# Autodesk Inventor assembly: LightRail_assembly
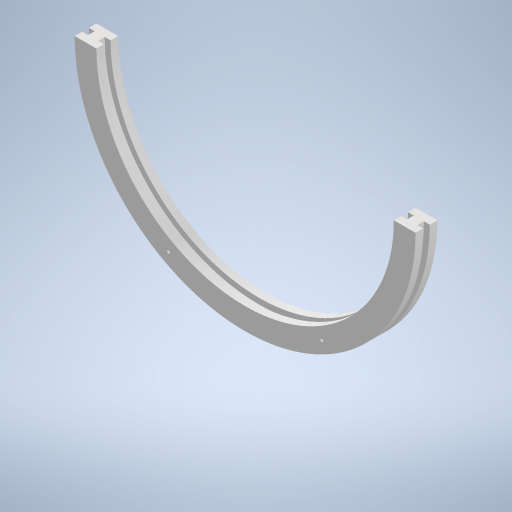
[picture p0: Inventor's stored thumbnail of the model, 512x512]
Saved by Autodesk Inventor 2023 (Build 270158000, 158)
## iProperties
Created: 2023-04-29
Part Number: LightRail_assembly
Document SubType Name: Assembly
Designer: ringl
Author: ringl
## Documents named in this file (3)
- C:\Users\ringl\Documents\Uni Classes\Y3S2\EE318-Project\EE318-Project\CAD\LightRail\LightRail_assembly.iam
- C:\Users\ringl\Documents\Uni Classes\Y3S2\EE318-Project\EE318-Project\CAD\LightRail\LightRail_endSection.ipt
- C:\Users\ringl\Documents\Uni Classes\Y3S2\EE318-Project\EE318-Project\CAD\LightRail\LightRail_middleSection.ipt
## Components (3 placed, 2 different names)
1. LightRail_endSection:1 — Mate:1, Mate:2, Flush:1
2. LightRail_middleSection:1 — Mate:1, Mate:2, Flush:1, Flush:2, Mate:3, Mate:4
3. LightRail_endSection:2 — Flush:2, Mate:3, Mate:4
## Relationships (6: Mate 4, Flush 2)
- Mate:1: LightRail_endSection:1 ↔ LightRail_middleSection:1
- Mate:2: LightRail_endSection:1 ↔ LightRail_middleSection:1
- Flush:1: LightRail_endSection:1 ↔ LightRail_middleSection:1
- Flush:2: LightRail_middleSection:1 ↔ LightRail_endSection:2
- Mate:3: LightRail_middleSection:1 ↔ LightRail_endSection:2
- Mate:4: LightRail_middleSection:1 ↔ LightRail_endSection:2
